# Autodesk Inventor assembly: Y_rail_Assembly_Rev3
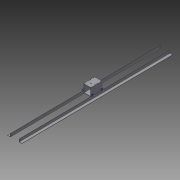
[picture p0: Inventor's stored thumbnail of the model, 180x180]
Saved by Autodesk Inventor 2015 (Build 190159000, 159)
## iProperties
Created: 2017-01-11
Part Number: Y_rail_Assembly_Rev3
Document SubType Name: Assembly
Designer: Guy
Mass: 1796.89 g
Surface Area: 4829.55 cm^2
Volume: 1200.62 cm^3
Density: 1.49664 g/cm^3
Author: Guy
## Documents named in this file (9)
- C:\Users\Guy\Documents\Fourth Year\Capstone\git\Capstone-Project\doc\CAD\LowLevel_Rev3\Y_rail_Assembly_Rev3.iam
- C:\Users\Guy\Documents\Fourth Year\Capstone\git\Capstone-Project\doc\CAD\LowLevel_Rev3\Y_Rail-SquareBar-Rev3.ipt
- C:\Users\Guy\Documents\Fourth Year\Capstone\git\Capstone-Project\doc\CAD\LowLevel_Rev3\XY_Wheel-SquareBar-Rev3.ipt
- C:\Users\Guy\Documents\Fourth Year\Capstone\git\Capstone-Project\doc\CAD\LowLevel_Rev3\Y_rail_Assembly_Rev3\Design Accelerator\Spur Gears1.iam
- C:\Users\Guy\Documents\Fourth Year\Capstone\git\Capstone-Project\doc\CAD\Stepper Motor\NEMA 17-old\M1173041- NEMA 17.ipt
- C:\Users\Guy\Documents\Fourth Year\Capstone\git\Capstone-Project\doc\CAD\Nuts and Bolts\3-16in_1 1-4in_Bolt.ipt
- C:\Users\Guy\Documents\Fourth Year\Capstone\git\Capstone-Project\doc\CAD\Nuts and Bolts\3-16in_7-16in_washer(num8).ipt
- C:\Users\Guy\Documents\Fourth Year\Capstone\git\Capstone-Project\doc\CAD\Nuts and Bolts\3-16in_1-16in_nut(num2).ipt
- C:\Users\Guy\Documents\Fourth Year\Capstone\git\Capstone-Project\doc\CAD\LowLevel_Rev3\EE_base\EE_base_assembly.iam
## Components (33 placed, 8 different names)
1. Y_Rail-SquareBar-Rev3:1 — Mate:39, Mate:97, Mate:99, Mate:102, Tangent:6
2. Y_Rail-SquareBar-Rev3:2 — Tangent:4, Mate:12, Mate:97, Mate:99, Mate:102, Tangent:5
3. XY_Wheel-SquareBar-Rev3:1 — Mate:9, Flush:2, Mate:39, Mate:45, Mate:51
4. XY_Wheel-SquareBar-Rev3:2 — Tangent:4, Mate:9, Flush:4, Mate:84, Mate:92, Mate:95, Mate:117
5. XY_Wheel-SquareBar-Rev3:3 — Mate:12, Flush:4, Mate:54, Mate:64, Mate:65, Tangent:5
6. XY_Wheel-SquareBar-Rev3:4 — Flush:2, Mate:73, Mate:79, Mate:80, Tangent:6
7. Spur Gears:1 [sub-assembly] — Mate:36, Flush:5, Mate:108
8. M1173041- NEMA 17:1 — Mate:36, Flush:5, Angle:2, Mate:118, Mate:119
9. 3-16in_1 1-4in_Bolt:1 — Mate:44, Mate:46, Mate:48, Mate:49, Mate:52, Mate:104, Mate:109
10. 3-16in_7-16in_washer(num8):3 — Mate:44, Mate:45, Mate:47
11. 3-16in_1-16in_nut(num2):1 — Mate:46, Mate:47
12. 3-16in_7-16in_washer(num8):4 — Mate:48, Mate:50, Mate:51
13. 3-16in_1-16in_nut(num2):2 — Mate:49, Mate:50
14. 3-16in_1-16in_nut(num2):3 — Mate:52, Mate:110
15. 3-16in_1 1-4in_Bolt:2 — Mate:54, Mate:56, Mate:57, Mate:58, Mate:59, Mate:60, Mate:106, Mate:113
16. 3-16in_1-16in_nut(num2):4 — Mate:56, Mate:61
17. 3-16in_1-16in_nut(num2):5 — Mate:58, Mate:114
18. 3-16in_1-16in_nut(num2):6 — Mate:59, Mate:62
19. 3-16in_7-16in_washer(num8):5 — Mate:57, Mate:62, Mate:64
20. 3-16in_7-16in_washer(num8):6 — Mate:60, Mate:61, Mate:65
21. 3-16in_1 1-4in_Bolt:3 — Mate:84, Mate:89, Mate:90, Mate:91, Mate:93, Mate:94, Mate:105, Mate:111
22. 3-16in_1 1-4in_Bolt:4 — Mate:73, Mate:75, Mate:77, Mate:78, Mate:82, Mate:83, Mate:107, Mate:115
23. 3-16in_1-16in_nut(num2):7 — Mate:86, Mate:91
24. 3-16in_1-16in_nut(num2):8 — Mate:87, Mate:94
25. 3-16in_1-16in_nut(num2):9 — Mate:89, Mate:112
26. 3-16in_1-16in_nut(num2):10 — Mate:76, Mate:78
27. 3-16in_1-16in_nut(num2):11 — Mate:81, Mate:82
28. 3-16in_1-16in_nut(num2):12 — Mate:75, Mate:116
29. 3-16in_7-16in_washer(num8):7 — Mate:80, Mate:81, Mate:83
30. 3-16in_7-16in_washer(num8):8 — Mate:87, Mate:93, Mate:95
31. 3-16in_7-16in_washer(num8):9 — Mate:76, Mate:77, Mate:79
32. 3-16in_7-16in_washer(num8):10 — Mate:86, Mate:90, Mate:92
33. EE_base_assembly:1 [sub-assembly] — Angle:2, Mate:104, Mate:105, Mate:106, Mate:107, Mate:108, Mate:109, Mate:110, Mate:111, Mate:112, Mate:113, Mate:114, Mate:115, Mate:116, Mate:117, Mate:118, Mate:119
## Relationships (69: Mate 62, Tangent 3, Flush 3, Angle 1)
- Tangent:4: Y_Rail-SquareBar-Rev3:2 ↔ XY_Wheel-SquareBar-Rev3:2
- Mate:9: XY_Wheel-SquareBar-Rev3:1 ↔ XY_Wheel-SquareBar-Rev3:2
- Flush:2: XY_Wheel-SquareBar-Rev3:1 ↔ XY_Wheel-SquareBar-Rev3:4
- Mate:12 (1.75 mm): Y_Rail-SquareBar-Rev3:2 ↔ XY_Wheel-SquareBar-Rev3:3
- Flush:4: XY_Wheel-SquareBar-Rev3:2 ↔ XY_Wheel-SquareBar-Rev3:3
- Mate:36: Spur Gears:1 ↔ M1173041- NEMA 17:1
- Flush:5 (-10 mm): Spur Gears:1 ↔ M1173041- NEMA 17:1
- Mate:39: Y_Rail-SquareBar-Rev3:1 ↔ XY_Wheel-SquareBar-Rev3:1
- Mate:44: 3-16in_1 1-4in_Bolt:1 ↔ 3-16in_7-16in_washer(num8):3
- Mate:45: XY_Wheel-SquareBar-Rev3:1 ↔ 3-16in_7-16in_washer(num8):3
- Mate:46: 3-16in_1 1-4in_Bolt:1 ↔ 3-16in_1-16in_nut(num2):1
- Mate:47: 3-16in_7-16in_washer(num8):3 ↔ 3-16in_1-16in_nut(num2):1
- Mate:48: 3-16in_1 1-4in_Bolt:1 ↔ 3-16in_7-16in_washer(num8):4
- Mate:49: 3-16in_1 1-4in_Bolt:1 ↔ 3-16in_1-16in_nut(num2):2
- Mate:50: 3-16in_7-16in_washer(num8):4 ↔ 3-16in_1-16in_nut(num2):2
- Mate:51: XY_Wheel-SquareBar-Rev3:1 ↔ 3-16in_7-16in_washer(num8):4
- Mate:52: 3-16in_1 1-4in_Bolt:1 ↔ 3-16in_1-16in_nut(num2):3
- Mate:54: XY_Wheel-SquareBar-Rev3:3 ↔ 3-16in_1 1-4in_Bolt:2
- Mate:56: 3-16in_1 1-4in_Bolt:2 ↔ 3-16in_1-16in_nut(num2):4
- Mate:57: 3-16in_1 1-4in_Bolt:2 ↔ 3-16in_7-16in_washer(num8):5
- Mate:58: 3-16in_1 1-4in_Bolt:2 ↔ 3-16in_1-16in_nut(num2):5
- Mate:59: 3-16in_1 1-4in_Bolt:2 ↔ 3-16in_1-16in_nut(num2):6
- Mate:60: 3-16in_1 1-4in_Bolt:2 ↔ 3-16in_7-16in_washer(num8):6
- Mate:61: 3-16in_1-16in_nut(num2):4 ↔ 3-16in_7-16in_washer(num8):6
- Mate:62: 3-16in_1-16in_nut(num2):6 ↔ 3-16in_7-16in_washer(num8):5
- Mate:64: XY_Wheel-SquareBar-Rev3:3 ↔ 3-16in_7-16in_washer(num8):5
- Mate:65: XY_Wheel-SquareBar-Rev3:3 ↔ 3-16in_7-16in_washer(num8):6
- Mate:73: XY_Wheel-SquareBar-Rev3:4 ↔ 3-16in_1 1-4in_Bolt:4
- Mate:75: 3-16in_1 1-4in_Bolt:4 ↔ 3-16in_1-16in_nut(num2):12
- Mate:76: 3-16in_1-16in_nut(num2):10 ↔ 3-16in_7-16in_washer(num8):9
- Mate:77: 3-16in_1 1-4in_Bolt:4 ↔ 3-16in_7-16in_washer(num8):9
- Mate:78: 3-16in_1 1-4in_Bolt:4 ↔ 3-16in_1-16in_nut(num2):10
- Mate:79: XY_Wheel-SquareBar-Rev3:4 ↔ 3-16in_7-16in_washer(num8):9
- Mate:80: XY_Wheel-SquareBar-Rev3:4 ↔ 3-16in_7-16in_washer(num8):7
- Mate:81: 3-16in_1-16in_nut(num2):11 ↔ 3-16in_7-16in_washer(num8):7
- Mate:82: 3-16in_1 1-4in_Bolt:4 ↔ 3-16in_1-16in_nut(num2):11
- Mate:83: 3-16in_1 1-4in_Bolt:4 ↔ 3-16in_7-16in_washer(num8):7
- Mate:84: XY_Wheel-SquareBar-Rev3:2 ↔ 3-16in_1 1-4in_Bolt:3
- Mate:86: 3-16in_1-16in_nut(num2):7 ↔ 3-16in_7-16in_washer(num8):10
- Mate:87: 3-16in_1-16in_nut(num2):8 ↔ 3-16in_7-16in_washer(num8):8
- Mate:89: 3-16in_1 1-4in_Bolt:3 ↔ 3-16in_1-16in_nut(num2):9
- Mate:90: 3-16in_1 1-4in_Bolt:3 ↔ 3-16in_7-16in_washer(num8):10
- Mate:91: 3-16in_1 1-4in_Bolt:3 ↔ 3-16in_1-16in_nut(num2):7
- Mate:92: XY_Wheel-SquareBar-Rev3:2 ↔ 3-16in_7-16in_washer(num8):10
- Mate:93: 3-16in_1 1-4in_Bolt:3 ↔ 3-16in_7-16in_washer(num8):8
- Mate:94: 3-16in_1 1-4in_Bolt:3 ↔ 3-16in_1-16in_nut(num2):8
- Mate:95: XY_Wheel-SquareBar-Rev3:2 ↔ 3-16in_7-16in_washer(num8):8
- Mate:97: Y_Rail-SquareBar-Rev3:1 ↔ Y_Rail-SquareBar-Rev3:2
- Mate:99 (95 mm): Y_Rail-SquareBar-Rev3:1 ↔ Y_Rail-SquareBar-Rev3:2
- Mate:102: Y_Rail-SquareBar-Rev3:1 ↔ Y_Rail-SquareBar-Rev3:2
- Tangent:5: Y_Rail-SquareBar-Rev3:2 ↔ XY_Wheel-SquareBar-Rev3:3
- Tangent:6: Y_Rail-SquareBar-Rev3:1 ↔ XY_Wheel-SquareBar-Rev3:4
- Angle:2 (0 deg): M1173041- NEMA 17:1 ↔ EE_base_assembly:1
- Mate:104: 3-16in_1 1-4in_Bolt:1 ↔ EE_base_assembly:1
- Mate:105: 3-16in_1 1-4in_Bolt:3 ↔ EE_base_assembly:1
- Mate:106: 3-16in_1 1-4in_Bolt:2 ↔ EE_base_assembly:1
- Mate:107: 3-16in_1 1-4in_Bolt:4 ↔ EE_base_assembly:1
- Mate:108: Spur Gears:1 ↔ EE_base_assembly:1
- Mate:109: 3-16in_1 1-4in_Bolt:1 ↔ EE_base_assembly:1
- Mate:110: 3-16in_1-16in_nut(num2):3 ↔ EE_base_assembly:1
- Mate:111: 3-16in_1 1-4in_Bolt:3 ↔ EE_base_assembly:1
- Mate:112: 3-16in_1-16in_nut(num2):9 ↔ EE_base_assembly:1
- Mate:113: 3-16in_1 1-4in_Bolt:2 ↔ EE_base_assembly:1
- Mate:114: 3-16in_1-16in_nut(num2):5 ↔ EE_base_assembly:1
- Mate:115: 3-16in_1 1-4in_Bolt:4 ↔ EE_base_assembly:1
- Mate:116: 3-16in_1-16in_nut(num2):12 ↔ EE_base_assembly:1
- Mate:117 (5.625 mm): XY_Wheel-SquareBar-Rev3:2 ↔ EE_base_assembly:1
- Mate:118: M1173041- NEMA 17:1 ↔ EE_base_assembly:1
- Mate:119 (15 mm): M1173041- NEMA 17:1 ↔ EE_base_assembly:1
